# Autodesk Inventor assembly: 000 Ensamblaje hw_DAA - PCB MicroSD
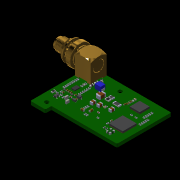
[picture p0: Inventor's stored thumbnail of the model, 180x180]
Saved by Autodesk Inventor 2018 (Build 220112000, 112)
## iProperties
Created: 2024-03-13
Part Number: 000 Ensamblaje hw_DAA - PCB MicroSD
Document SubType Name: Assembly
Designer: cda1
Author: cda1
## Documents named in this file (48)
- C:\Users\cda1\Git\DAA\items\hw_DAA\variants\BASIC\3d\000 Ensamblaje hw_DAA - PCB MicroSD.iam
- C:\Users\cda1\Git\DAA\items\hw_DAA\3d\hw_DAA - PCB MicroSD.ipt
- C:\Users\cda1\Git\DAA\items\_accessories\Componentes PCB\Tarjetero\3d_Molex\3d\47219-2001.ipt
- C:\Users\cda1\Git\DAA\items\_accessories\Cables y conectores\3d_Amphenol\3d\132203-18\132203-18.ipt
- C:\Users\cda1\Git\DAA\items\_accessories\Componentes PCB\PMIC\TPS65033000RGERQ1\TPS65033000RGERQ1.iam
- C:\Users\cda1\Git\DAA\items\_accessories\Componentes PCB\Inductor\3d_TDK\3d\NLCV32T-100K-EFRD\NLCV32T-100K-EFRD.iam
- C:\Users\cda1\Git\DAA\items\_accessories\Componentes PCB\Ferrita\3d_Murata Electronics\3d\BLM18SG121TN1D\BLM18SG121TN1D.ipt
- C:\Users\cda1\Git\DAA\items\_accessories\Componentes PCB\EMI Suppressor\3d_Murata_Electronics\BLM18AG102BH1D\BLM18AG102BH1D.ipt
- C:\Users\cda1\Git\DAA\items\_accessories\Componentes PCB\EMI Suppressor\3d_Murata_Electronics\BLM18HE152SZ1D\BLM18HE152SZ1D.ipt
- C:\Users\cda1\Git\DAA\items\_accessories\Componentes PCB\MIPI\DS90UB953TRHBTQ1\DS90UB953TRHBTQ1.iam
- C:\Users\cda1\Git\DAA\items\_accessories\Componentes PCB\FPD-Link\3d_Texas_Instruments\DS90UB954TRGZTQ1\DS90UB954TRGZTQ1.iam
- C:\Users\cda1\Git\DAA\items\_accessories\Componentes PCB\Oscilador\3d_ECS_International\ECS-2520MVQ-250-CN-TR\ECS-2520MVQ-250-CN-TR.ipt
- C:\Users\cda1\Git\DAA\items\_accessories\Componentes PCB\Capacitadores\3d_TDK\3d\CGA5L1X7R1V106K160AC.ipt
- C:\Users\cda1\Git\DAA\items\_accessories\Componentes PCB\Capacitadores\3d_TDK\3d\CGA2B3X7R1H104K050BD.ipt
- C:\Users\cda1\Git\DAA\items\_accessories\Componentes PCB\Capacitadores\3d_Taiyo Yuden\3d\EMK212BBJ106KGHT.ipt
- C:\Users\cda1\Git\DAA\items\_accessories\Componentes PCB\Resistencias\3d_Panasonic\3d\ERJ-2RKF1002X.ipt
- C:\Users\cda1\Git\DAA\items\_accessories\Componentes PCB\Resistencias\3d_Yageo\3d\AC1206FR-074R02L\AC1206FR-074R02L.ipt
- C:\Users\cda1\Git\DAA\items\_accessories\Componentes PCB\Resistencias\3d_Yageo\3d\AC0805FR-070RL.ipt
- C:\Users\cda1\Git\DAA\items\_accessories\Componentes PCB\Capacitadores\3d_Murata Electronics\3d\GRT188C81A106ME13D\GRT188C81A106ME13D.iam
- C:\Users\cda1\Git\DAA\items\_accessories\Componentes PCB\Capacitadores\3d_TDK\3d\CGA2B3X8R1H103K050BB.ipt
- C:\Users\cda1\Git\DAA\items\_accessories\Componentes PCB\Voltage-Level\3d\3d_NXP\NVT4858HK\NVT4858HK.ipt
- C:\Users\cda1\Git\DAA\items\_accessories\Componentes PCB\ESD Supressor\3d_Littlefuse\3d\AQ4020-01FTG\AQ4020-01FTG.iam
- C:\Users\cda1\Git\DAA\items\_accessories\Componentes PCB\Active-low load\3d_Texas_Instruments\TPS22910AYZVR\TPS22910AYZVR.iam
- C:\Users\cda1\Git\DAA\items\_accessories\Componentes PCB\Capacitadores\3d_Murata Electronics\3d\GRT155R61E105KE01D.ipt
- C:\Users\cda1\Git\DAA\items\_accessories\Componentes PCB\Inverter\3d_Texas Instruments\3d\SN74LVC1G04QDCKRQ1\SN74LVC1G04QDCKRQ1.iam
- C:\Users\cda1\Git\DAA\items\_accessories\Componentes PCB\Capacitadores\3d_Murata Electronics\3d\NFM18HC106D0G3L\NFM18HC106D0G3L.ipt
- C:\Users\cda1\Git\DAA\items\_accessories\Componentes PCB\Capacitadores\3d_TDK\3d\CGA3E1X7S1C225K080AC\CGA3E1X7S1C225K080AC.iam
- C:\Users\cda1\Git\DAA\items\_accessories\Componentes PCB\Resistencias\3d_Panasonic\3d\ERJ-2GE0R00X.ipt
- C:\Users\cda1\Git\DAA\items\_accessories\Componentes PCB\Capacitadores\3d_Murata Electronics\3d\GCM155R71H153KA55D\GCM155R71H153KA55D.iam
- C:\Users\cda1\Git\DAA\items\_accessories\Componentes PCB\Resistencias\3d_Panasonic\3d\ERJ-U02F4701X\ERJ-U02F4701X.iam
- C:\Users\cda1\Git\DAA\items\_accessories\Componentes PCB\Capacitadores\3d_Kemet\3d\C0402C223K5RECAUTO.ipt
- C:\Users\cda1\Git\DAA\items\_accessories\Componentes PCB\Capacitadores\3d_TDK\3d\CGA2B3X7R1H333K050BB.ipt
- C:\Users\cda1\Git\DAA\items\_accessories\Componentes PCB\Resistencias\3d_Vishay\3d\CRCW040249R9FKED\CRCW040249R9FKED.ipt
- C:\Users\cda1\Git\DAA\items\_accessories\Componentes PCB\Condensadores\3d-Murata\3d\GRT155R61A475ME13D\GRT155R61A475ME13D.iam
- C:\Users\cda1\Git\DAA\items\_accessories\Componentes PCB\Condensadores\3d-Murata\3d\GRT155C81C225KE13D.ipt
- C:\Users\cda1\Git\DAA\items\_accessories\Componentes PCB\Resistencias\3d_Vishay\3d\CRCW040240K2FKED\CRCW040240K2FKED.ipt
- C:\Users\cda1\Git\DAA\items\_accessories\Componentes PCB\Capacitadores\3d_Taiyo Yuden\3d\HMJ107BB7104KAHT.ipt
- C:\Users\cda1\Git\DAA\items\_accessories\Componentes PCB\Resistencias\3d_Genérico\RESC-1206.ipt
- C:\Users\cda1\Git\DAA\items\_accessories\Componentes PCB\Diodos\3d_Diodes Incorporated\3d\DMN2710UTQ-7\DMN2710UTQ-7.ipt
- C:\Users\cda1\Git\DAA\items\_accessories\Componentes PCB\Inductor\3d_TDK\3d\TFM201610ALMA1R0MTAA\TFM201610ALMA1R0MTAA.iam
- C:\Users\cda1\Git\DAA\items\_accessories\Componentes PCB\Inductor\3d_TDK\3d\TFM201610ALMA1R5MTAA\TFM201610ALMA1R5MTAA.iam
- C:\Users\cda1\Git\DAA\items\_accessories\Componentes PCB\Resistencias\3d_Genérico\RESC-0402.ipt
- C:\Users\cda1\Git\DAA\items\_accessories\Componentes PCB\Diodos\3d_TE_Connectivity\3d\PESD0402-140\PESD0402-140.iam
- C:\Users\cda1\Git\DAA\items\_accessories\Componentes PCB\Resistencias\3d_Genérico\RESC-0603.ipt
- C:\Users\cda1\Git\DAA\items\_accessories\Componentes PCB\Capacitadores\3d_Genérico\3d\CAPC-0402-T0.55-BN.ipt
- C:\Users\cda1\Git\DAA\items\_accessories\Componentes PCB\Transistores\3d_Diodes\3d\DMP2006UFGQ-13\DMP2006UFGQ-13.iam
- C:\Users\cda1\Git\DAA\items\_accessories\Componentes PCB\Resistencias\3d_Panasonic\3d\ERJ-2RKF33R0X.ipt
- C:\Users\cda1\Git\DAA\items\_accessories\Componentes PCB\Resistencias\3d_Genérico\RESC-0805.ipt
## Components (182 placed, 47 different names)
1. hw_DAA - PCB MicroSD:1 — Coincidencia:3, Coincidencia:4, Coincidencia:9, Coincidencia:14, Coincidencia:17, Coincidencia:18, Coincidencia:20, Coincidencia:24, Coincidencia:25, Coincidencia:34, Coincidencia:35, Coincidencia:36, Coincidencia:38, Coincidencia:39, Coincidencia:40, Coincidencia:42, Coincidencia:43, Coincidencia:50, Coincidencia:51, Coincidencia:52, Coincidencia:53, Coincidencia:54, Coincidencia:55, Coincidencia:56, Coincidencia:57, Coincidencia:59, Coincidencia:60, Coincidencia:62, Coincidencia:63, Coincidencia:64, Coincidencia:65, Coincidencia:67, Coincidencia:69, Coincidencia:70, Coincidencia:71, Coincidencia:72, Coincidencia:73, Coincidencia:74, Coincidencia:75, Coincidencia:76, Coincidencia:79, Coincidencia:95, Coincidencia:96, Coincidencia:97, Coincidencia:99, Coincidencia:101, Coincidencia:102, Coincidencia:117, Coincidencia:130, Coincidencia:131, Coincidencia:132, Coincidencia:133, Coincidencia:134, Coincidencia:135, Coincidencia:137, Coincidencia:138, Coincidencia:140, Coincidencia:141, Coincidencia:155, Coincidencia:156, Coincidencia:157, Coincidencia:158, Coincidencia:159, Coincidencia:165, Coincidencia:166, Coincidencia:167, Coincidencia:182, Coincidencia:183, Coincidencia:186, Coincidencia:187, Coincidencia:189, Coincidencia:190, Coincidencia:191, Coincidencia:192, Coincidencia:193, Coincidencia:194, Coincidencia:197, Coincidencia:198, Coincidencia:199, Coincidencia:204, Coincidencia:205, Coincidencia:206, Coincidencia:207, Coincidencia:208, Coincidencia:209, Coincidencia:210, Coincidencia:211, Ángulo:3, Ángulo:4, Coincidencia:212, Coincidencia:213, Coincidencia:214, Coincidencia:215, Coincidencia:216, Coincidencia:217, Coincidencia:218, Coincidencia:219, Coincidencia:220, Ángulo:6, Coincidencia:221, Ángulo:7, Coincidencia:222, Coincidencia:223, Ángulo:8, Ángulo:9, Coincidencia:224, Coincidencia:225, Coincidencia:226, Coincidencia:227, Coincidencia:228, Coincidencia:229, Coincidencia:230, Coincidencia:231, Coincidencia:232, Coincidencia:233, Coincidencia:234, Coincidencia:235, Coincidencia:236, Coincidencia:237, Coincidencia:238, Coincidencia:240, Coincidencia:241, Coincidencia:244, Coincidencia:245, Coincidencia:246, Coincidencia:249, Coincidencia:250, Coincidencia:251, Coincidencia:252, Coincidencia:253, Coincidencia:254, Coincidencia:255, Coincidencia:256, Coincidencia:257, Coincidencia:258, Coincidencia:259, Coincidencia:260, Coincidencia:261, Coincidencia:262, Coincidencia:263, Coincidencia:264, Coincidencia:265, Ángulo:11, Coincidencia:266, Coincidencia:267, Coincidencia:268, Coincidencia:269, Ángulo:12, Ángulo:13, Coincidencia:270, Coincidencia:271, Ángulo:16, Coincidencia:272, Coincidencia:273, Coincidencia:274, Coincidencia:275, Coincidencia:276, Coincidencia:277, Coincidencia:278, Coincidencia:279, Coincidencia:280, Coincidencia:281, Coincidencia:282, Coincidencia:283, Coincidencia:284, Coincidencia:285, Ángulo:17, Coincidencia:286, Coincidencia:287, Ángulo:18, Ángulo:19, Coincidencia:288, Coincidencia:289, Coincidencia:290, Coincidencia:291, Coincidencia:292, Coincidencia:293, Coincidencia:294, Coincidencia:295, Coincidencia:296, Coincidencia:297, Coincidencia:298, Coincidencia:299, Coincidencia:300, Coincidencia:301, Coincidencia:302, Coincidencia:303, Coincidencia:304, Coincidencia:305, Coincidencia:306, Coincidencia:307, Coincidencia:308, Coincidencia:309, Coincidencia:310, Coincidencia:311
2. 47219-2001:1 — Coincidencia:182
3. 132203-18:1 — Coincidencia:3, Coincidencia:271, Ángulo:16
4. TPS65033000RGERQ1:1 [sub-assembly] — Coincidencia:4
5. NLCV32T-100K-EFRD:1 [sub-assembly] — Coincidencia:263
6. BLM18SG121TN1D:1 — Coincidencia:9
7. BLM18AG102BH1D:2 — Coincidencia:14
8. BLM18AG102BH1D:4 — Coincidencia:17
9. BLM18AG102BH1D:5 — Coincidencia:18
10. BLM18AG102BH1D:7 — Coincidencia:20
11. BLM18HE152SZ1D:1
12. BLM18HE152SZ1D:2 — Coincidencia:268
13. BLM18HE152SZ1D:3 — Coincidencia:267
14. DS90UB953TRHBTQ1:1 [sub-assembly] — Coincidencia:24
15. DS90UB954TRGZTQ1:1 [sub-assembly] — Coincidencia:25
16. CGA5L1X7R1V106K160AC:1 — Coincidencia:264, Ángulo:17
17. CGA5L1X7R1V106K160AC:2 — Coincidencia:34
18. CGA5L1X7R1V106K160AC:3 — Coincidencia:35
19. CGA2B3X7R1H104K050BD:1 — Coincidencia:36
20. CGA2B3X7R1H104K050BD:4 — Coincidencia:39
21. CGA2B3X7R1H104K050BD:5 — Coincidencia:40
22. CGA2B3X7R1H104K050BD:6 — Coincidencia:38
23. CGA2B3X7R1H104K050BD:7 — Coincidencia:42
24. CGA2B3X7R1H104K050BD:8 — Coincidencia:43
25. CGA2B3X7R1H104K050BD:15 — Coincidencia:50
26. CGA2B3X7R1H104K050BD:16 — Coincidencia:51
27. CGA2B3X7R1H104K050BD:17 — Coincidencia:53
28. CGA2B3X7R1H104K050BD:18 — Coincidencia:52
29. CGA2B3X7R1H104K050BD:19 — Coincidencia:54
30. CGA2B3X7R1H104K050BD:20 — Coincidencia:55
31. CGA2B3X7R1H104K050BD:21 — Coincidencia:56
32. CGA2B3X7R1H104K050BD:22 — Coincidencia:57
33. CGA2B3X7R1H104K050BD:24 — Coincidencia:60
34. CGA2B3X7R1H104K050BD:25 — Coincidencia:59
35. CGA2B3X7R1H104K050BD:28 — Coincidencia:65
36. CGA2B3X7R1H104K050BD:29 — Coincidencia:64
37. CGA2B3X7R1H104K050BD:30 — Coincidencia:63
38. CGA2B3X7R1H104K050BD:31 — Coincidencia:62
39. CGA2B3X7R1H104K050BD:32 — Coincidencia:72
40. CGA2B3X7R1H104K050BD:33 — Coincidencia:71
41. CGA2B3X7R1H104K050BD:34 — Coincidencia:70
42. CGA2B3X7R1H104K050BD:35 — Coincidencia:69
43. CGA2B3X7R1H104K050BD:37 — Coincidencia:67
44. CGA2B3X7R1H104K050BD:38 — Coincidencia:76
45. CGA2B3X7R1H104K050BD:39 — Coincidencia:75
46. CGA2B3X7R1H104K050BD:40 — Coincidencia:74
47. CGA2B3X7R1H104K050BD:41 — Coincidencia:73
48. CGA2B3X7R1H104K050BD:44 — Coincidencia:79
49. CGA2B3X7R1H104K050BD:55 — Coincidencia:95
50. CGA2B3X7R1H104K050BD:56 — Coincidencia:96
51. CGA2B3X7R1H104K050BD:57 — Coincidencia:97
52. CGA2B3X7R1H104K050BD:59 — Coincidencia:99
53. CGA2B3X7R1H104K050BD:61 — Coincidencia:101
54. CGA2B3X7R1H104K050BD:62 — Coincidencia:102
55. EMK212BBJ106KGHT:1 — Coincidencia:186
56. EMK212BBJ106KGHT:2 — Coincidencia:187
57. EMK212BBJ106KGHT:3 — Coincidencia:286
58. ERJ-2RKF1002X:1 — Coincidencia:117
59. ERJ-2RKF1002X:14 — Coincidencia:130
60. ERJ-2RKF1002X:15 — Coincidencia:131
61. ERJ-2RKF1002X:16 — Coincidencia:132
62. ERJ-2RKF1002X:17 — Coincidencia:133
63. ERJ-2RKF1002X:18 — Coincidencia:134
64. ERJ-2RKF1002X:19 — Coincidencia:135
65. ERJ-2RKF1002X:21 — Coincidencia:137
66. ERJ-2RKF1002X:22 — Coincidencia:138
67. ERJ-2RKF1002X:24 — Coincidencia:140
68. ERJ-2RKF1002X:25 — Coincidencia:141
69. ERJ-2RKF1002X:38
70. ERJ-2RKF1002X:39 — Coincidencia:155
71. ERJ-2RKF1002X:40 — Coincidencia:158
72. ERJ-2RKF1002X:41 — Coincidencia:159
73. ERJ-2RKF1002X:42 — Coincidencia:156
74. ERJ-2RKF1002X:43 — Coincidencia:157
75. ERJ-2RKF1002X:49 — Coincidencia:165
76. ERJ-2RKF1002X:50 — Coincidencia:166
77. ERJ-2RKF1002X:51 — Coincidencia:167
78. CGA5L1X7R1V106K160AC:4 — Coincidencia:183, Ángulo:13
79. AC1206FR-074R02L:1 — Coincidencia:262
80. AC0805FR-070RL:1 — Coincidencia:266
81. EMK212BBJ106KGHT:4 — Coincidencia:189
82. GRT188C81A106ME13D:1 [sub-assembly] — Coincidencia:190
83. GRT188C81A106ME13D:2 [sub-assembly] — Coincidencia:191
84. GRT188C81A106ME13D:3 [sub-assembly] — Coincidencia:192
85. GRT188C81A106ME13D:4 [sub-assembly] — Coincidencia:193
86. GRT188C81A106ME13D:5 [sub-assembly] — Coincidencia:194
87. CGA2B3X8R1H103K050BB:1 — Coincidencia:197
88. CGA2B3X8R1H103K050BB:2 — Coincidencia:198
89. GRT188C81A106ME13D:6 [sub-assembly] — Coincidencia:199
90. NVT4858HK:1 — Coincidencia:204
91. AQ4020-01FTG:1 [sub-assembly] — Coincidencia:205
92. TPS22910AYZVR:1 [sub-assembly] — Coincidencia:206
93. TPS22910AYZVR:2 [sub-assembly] — Coincidencia:207
94. GRT155R61E105KE01D:1 — Coincidencia:208
95. GRT188C81A106ME13D:7 [sub-assembly] — Coincidencia:209
96. SN74LVC1G04QDCKRQ1:1 [sub-assembly] — Coincidencia:210, Coincidencia:211
97. NFM18HC106D0G3L:1 — Ángulo:3, Coincidencia:212
98. NFM18HC106D0G3L:2 — Ángulo:4, Coincidencia:213
99. EMK212BBJ106KGHT:5 — Coincidencia:215
100. EMK212BBJ106KGHT:6 — Coincidencia:214
101. CGA3E1X7S1C225K080AC:1 [sub-assembly] — Coincidencia:216, Ángulo:5
102. GRT155R61E105KE01D:2 — Coincidencia:217
103. CGA3E1X7S1C225K080AC:2 [sub-assembly] — Coincidencia:218, Ángulo:5
104. ERJ-2GE0R00X:1 — Coincidencia:219
105. ERJ-2GE0R00X:2 — Coincidencia:220, Ángulo:6
106. GCM155R71H153KA55D:1 [sub-assembly] — Coincidencia:221, Ángulo:7
107. ERJ-U02F4701X:1 [sub-assembly] — Coincidencia:222, Ángulo:9
108. ERJ-U02F4701X:2 [sub-assembly] — Coincidencia:223, Ángulo:8
109. ECS-2520MVQ-250-CN-TR:2 — Coincidencia:224
110. GCM155R71H153KA55D:2 [sub-assembly] — Coincidencia:225
111. CGA2B3X7R1H104K050BD:68 — Coincidencia:226
112. C0402C223K5RECAUTO:1 — Coincidencia:227
113. C0402C223K5RECAUTO:2 — Coincidencia:228
114. CGA2B3X7R1H333K050BB:1 — Coincidencia:229
115. CGA2B3X7R1H333K050BB:2 — Coincidencia:230
116. CRCW040249R9FKED:1 — Coincidencia:231
117. GRT155R61E105KE01D:3 — Coincidencia:232
118. GRT155R61E105KE01D:4 — Coincidencia:233
119. GRT155R61A475ME13D:1 [sub-assembly] — Coincidencia:234
120. CGA2B3X7R1H104K050BD:69 — Coincidencia:235
121. ERJ-2RKF1002X:65 — Coincidencia:236, Ángulo:18
122. GRT155C81C225KE13D:1 — Coincidencia:237, Ángulo:19
123. ERJ-2RKF1002X:66 — Coincidencia:238
124. BLM18AG102BH1D:8 — Coincidencia:240
125. CRCW040240K2FKED:1 — Coincidencia:241
126. ERJ-2GE0R00X:3 — Coincidencia:244
127. ERJ-2GE0R00X:4 — Coincidencia:246
128. ERJ-2GE0R00X:5 — Coincidencia:245
129. HMJ107BB7104KAHT:1 — Coincidencia:265, Ángulo:11
130. DMN2710UTQ-7:1 — Coincidencia:249, Coincidencia:250
131. TFM201610ALMA1R0MTAA:1 [sub-assembly] — Coincidencia:251
132. TFM201610ALMA1R5MTAA:1 [sub-assembly] — Coincidencia:252
133. TFM201610ALMA1R0MTAA:2 [sub-assembly] — Coincidencia:253
134. CGA2B3X7R1H104K050BD:70 — Coincidencia:254
135. RESC-0402:1 — Coincidencia:255
136. RESC-0402:2 — Coincidencia:256
137. ERJ-2RKF1002X:67 — Coincidencia:257
138. PESD0402-140:1 [sub-assembly] — Coincidencia:258
139. RESC-0603:1 — Coincidencia:259
140. CAPC-0402-T0.55-BN:1 — Coincidencia:260
141. RESC-0402:3 — Coincidencia:261
142. RESC-1206:2 — Coincidencia:269, Ángulo:12
143. DMP2006UFGQ-13:1 [sub-assembly] — Coincidencia:270
144. ERJ-2RKF33R0X:1 — Coincidencia:272
145. ERJ-2RKF33R0X:2 — Coincidencia:273
146. ERJ-2RKF33R0X:3 — Coincidencia:274
147. ERJ-2RKF33R0X:4 — Coincidencia:275
148. ERJ-2RKF33R0X:5 — Coincidencia:277
149. ERJ-2RKF33R0X:6 — Coincidencia:278
150. ERJ-2RKF33R0X:7 — Coincidencia:279
151. ERJ-2RKF33R0X:8 — Coincidencia:281
152. ERJ-2RKF33R0X:9 — Coincidencia:282
153. ERJ-2RKF33R0X:10 — Coincidencia:283
154. ERJ-2RKF33R0X:11 — Coincidencia:284
155. ERJ-2RKF33R0X:12 — Coincidencia:285
156. ERJ-2RKF33R0X:13 — Coincidencia:280
157. ERJ-2RKF33R0X:14 — Coincidencia:276
158. RESC-0805:1 — Coincidencia:287
159. ERJ-2RKF1002X:68 — Coincidencia:288
160. ERJ-2RKF1002X:69 — Coincidencia:289
161. ERJ-2RKF1002X:70 — Coincidencia:290
162. ERJ-2RKF1002X:71 — Coincidencia:291
163. ERJ-2RKF1002X:72 — Coincidencia:292
164. ERJ-2RKF1002X:73 — Coincidencia:293
165. ERJ-2RKF1002X:74 — Coincidencia:294
166. ERJ-2RKF1002X:75 — Coincidencia:295
167. ERJ-2RKF1002X:76 — Coincidencia:296
168. ERJ-2RKF1002X:77 — Coincidencia:297
169. ERJ-2RKF1002X:78 — Coincidencia:298
170. ERJ-2RKF1002X:79 — Coincidencia:299
171. ERJ-2GE0R00X:6 — Coincidencia:300
172. ERJ-2GE0R00X:7 — Coincidencia:301
173. ERJ-2GE0R00X:8 — Coincidencia:302
174. ERJ-2GE0R00X:9 — Coincidencia:303
175. ERJ-2GE0R00X:10 — Coincidencia:304
176. ERJ-2GE0R00X:11 — Coincidencia:305
177. ERJ-2GE0R00X:12 — Coincidencia:306
178. ERJ-2GE0R00X:13 — Coincidencia:307
179. ERJ-2GE0R00X:14 — Coincidencia:308
180. ERJ-2GE0R00X:15 — Coincidencia:309
181. ERJ-2GE0R00X:16 — Coincidencia:310
182. ERJ-2GE0R00X:17 — Coincidencia:311
## Relationships (196: Mate 182, Angle 14)
- Coincidencia:3 [Mate]: hw_DAA - PCB MicroSD:1 ↔ 132203-18:1
- Coincidencia:4 [Mate]: hw_DAA - PCB MicroSD:1 ↔ TPS65033000RGERQ1:1
- Coincidencia:9 [Mate]: hw_DAA - PCB MicroSD:1 ↔ BLM18SG121TN1D:1
- Coincidencia:14 [Mate]: hw_DAA - PCB MicroSD:1 ↔ BLM18AG102BH1D:2
- Coincidencia:17 [Mate]: hw_DAA - PCB MicroSD:1 ↔ BLM18AG102BH1D:4
- Coincidencia:18 [Mate]: hw_DAA - PCB MicroSD:1 ↔ BLM18AG102BH1D:5
- Coincidencia:20 [Mate]: hw_DAA - PCB MicroSD:1 ↔ BLM18AG102BH1D:7
- Coincidencia:24 [Mate]: hw_DAA - PCB MicroSD:1 ↔ DS90UB953TRHBTQ1:1
- Coincidencia:25 [Mate]: hw_DAA - PCB MicroSD:1 ↔ DS90UB954TRGZTQ1:1
- Coincidencia:34 [Mate]: hw_DAA - PCB MicroSD:1 ↔ CGA5L1X7R1V106K160AC:2
- Coincidencia:35 [Mate]: hw_DAA - PCB MicroSD:1 ↔ CGA5L1X7R1V106K160AC:3
- Coincidencia:36 [Mate]: hw_DAA - PCB MicroSD:1 ↔ CGA2B3X7R1H104K050BD:1
- Coincidencia:38 [Mate]: hw_DAA - PCB MicroSD:1 ↔ CGA2B3X7R1H104K050BD:6
- Coincidencia:39 [Mate]: hw_DAA - PCB MicroSD:1 ↔ CGA2B3X7R1H104K050BD:4
- Coincidencia:40 [Mate]: hw_DAA - PCB MicroSD:1 ↔ CGA2B3X7R1H104K050BD:5
- Coincidencia:42 [Mate]: hw_DAA - PCB MicroSD:1 ↔ CGA2B3X7R1H104K050BD:7
- Coincidencia:43 [Mate]: hw_DAA - PCB MicroSD:1 ↔ CGA2B3X7R1H104K050BD:8
- Coincidencia:50 [Mate]: hw_DAA - PCB MicroSD:1 ↔ CGA2B3X7R1H104K050BD:15
- Coincidencia:51 [Mate]: hw_DAA - PCB MicroSD:1 ↔ CGA2B3X7R1H104K050BD:16
- Coincidencia:52 [Mate]: hw_DAA - PCB MicroSD:1 ↔ CGA2B3X7R1H104K050BD:18
- Coincidencia:53 [Mate]: hw_DAA - PCB MicroSD:1 ↔ CGA2B3X7R1H104K050BD:17
- Coincidencia:54 [Mate]: hw_DAA - PCB MicroSD:1 ↔ CGA2B3X7R1H104K050BD:19
- Coincidencia:55 [Mate]: hw_DAA - PCB MicroSD:1 ↔ CGA2B3X7R1H104K050BD:20
- Coincidencia:56 [Mate]: hw_DAA - PCB MicroSD:1 ↔ CGA2B3X7R1H104K050BD:21
- Coincidencia:57 [Mate]: hw_DAA - PCB MicroSD:1 ↔ CGA2B3X7R1H104K050BD:22
- Coincidencia:59 [Mate]: hw_DAA - PCB MicroSD:1 ↔ CGA2B3X7R1H104K050BD:25
- Coincidencia:60 [Mate]: hw_DAA - PCB MicroSD:1 ↔ CGA2B3X7R1H104K050BD:24
- Coincidencia:62 [Mate]: hw_DAA - PCB MicroSD:1 ↔ CGA2B3X7R1H104K050BD:31
- Coincidencia:63 [Mate]: hw_DAA - PCB MicroSD:1 ↔ CGA2B3X7R1H104K050BD:30
- Coincidencia:64 [Mate]: hw_DAA - PCB MicroSD:1 ↔ CGA2B3X7R1H104K050BD:29
- Coincidencia:65 [Mate]: hw_DAA - PCB MicroSD:1 ↔ CGA2B3X7R1H104K050BD:28
- Coincidencia:67 [Mate]: hw_DAA - PCB MicroSD:1 ↔ CGA2B3X7R1H104K050BD:37
- Coincidencia:69 [Mate]: hw_DAA - PCB MicroSD:1 ↔ CGA2B3X7R1H104K050BD:35
- Coincidencia:70 [Mate]: hw_DAA - PCB MicroSD:1 ↔ CGA2B3X7R1H104K050BD:34
- Coincidencia:71 [Mate]: hw_DAA - PCB MicroSD:1 ↔ CGA2B3X7R1H104K050BD:33
- Coincidencia:72 [Mate]: hw_DAA - PCB MicroSD:1 ↔ CGA2B3X7R1H104K050BD:32
- Coincidencia:73 [Mate]: hw_DAA - PCB MicroSD:1 ↔ CGA2B3X7R1H104K050BD:41
- Coincidencia:74 [Mate]: hw_DAA - PCB MicroSD:1 ↔ CGA2B3X7R1H104K050BD:40
- Coincidencia:75 [Mate]: hw_DAA - PCB MicroSD:1 ↔ CGA2B3X7R1H104K050BD:39
- Coincidencia:76 [Mate]: hw_DAA - PCB MicroSD:1 ↔ CGA2B3X7R1H104K050BD:38
- Coincidencia:79 [Mate]: hw_DAA - PCB MicroSD:1 ↔ CGA2B3X7R1H104K050BD:44
- Coincidencia:95 [Mate]: hw_DAA - PCB MicroSD:1 ↔ CGA2B3X7R1H104K050BD:55
- Coincidencia:96 [Mate]: hw_DAA - PCB MicroSD:1 ↔ CGA2B3X7R1H104K050BD:56
- Coincidencia:97 [Mate]: hw_DAA - PCB MicroSD:1 ↔ CGA2B3X7R1H104K050BD:57
- Coincidencia:99 [Mate]: hw_DAA - PCB MicroSD:1 ↔ CGA2B3X7R1H104K050BD:59
- Coincidencia:101 [Mate]: hw_DAA - PCB MicroSD:1 ↔ CGA2B3X7R1H104K050BD:61
- Coincidencia:102 [Mate]: hw_DAA - PCB MicroSD:1 ↔ CGA2B3X7R1H104K050BD:62
- Coincidencia:117 [Mate]: hw_DAA - PCB MicroSD:1 ↔ ERJ-2RKF1002X:1
- Coincidencia:130 [Mate]: hw_DAA - PCB MicroSD:1 ↔ ERJ-2RKF1002X:14
- Coincidencia:131 [Mate]: hw_DAA - PCB MicroSD:1 ↔ ERJ-2RKF1002X:15
- Coincidencia:132 [Mate]: hw_DAA - PCB MicroSD:1 ↔ ERJ-2RKF1002X:16
- Coincidencia:133 [Mate]: hw_DAA - PCB MicroSD:1 ↔ ERJ-2RKF1002X:17
- Coincidencia:134 [Mate]: hw_DAA - PCB MicroSD:1 ↔ ERJ-2RKF1002X:18
- Coincidencia:135 [Mate]: hw_DAA - PCB MicroSD:1 ↔ ERJ-2RKF1002X:19
- Coincidencia:137 [Mate]: hw_DAA - PCB MicroSD:1 ↔ ERJ-2RKF1002X:21
- Coincidencia:138 [Mate]: hw_DAA - PCB MicroSD:1 ↔ ERJ-2RKF1002X:22
- Coincidencia:140 [Mate]: hw_DAA - PCB MicroSD:1 ↔ ERJ-2RKF1002X:24
- Coincidencia:141 [Mate]: hw_DAA - PCB MicroSD:1 ↔ ERJ-2RKF1002X:25
- Coincidencia:155 [Mate]: hw_DAA - PCB MicroSD:1 ↔ ERJ-2RKF1002X:39
- Coincidencia:156 [Mate]: hw_DAA - PCB MicroSD:1 ↔ ERJ-2RKF1002X:42
- Coincidencia:157 [Mate]: hw_DAA - PCB MicroSD:1 ↔ ERJ-2RKF1002X:43
- Coincidencia:158 [Mate]: hw_DAA - PCB MicroSD:1 ↔ ERJ-2RKF1002X:40
- Coincidencia:159 [Mate]: hw_DAA - PCB MicroSD:1 ↔ ERJ-2RKF1002X:41
- Coincidencia:165 [Mate]: hw_DAA - PCB MicroSD:1 ↔ ERJ-2RKF1002X:49
- Coincidencia:166 [Mate]: hw_DAA - PCB MicroSD:1 ↔ ERJ-2RKF1002X:50
- Coincidencia:167 [Mate]: hw_DAA - PCB MicroSD:1 ↔ ERJ-2RKF1002X:51
- Coincidencia:182 [Mate]: hw_DAA - PCB MicroSD:1 ↔ 47219-2001:1
- Coincidencia:183 [Mate]: hw_DAA - PCB MicroSD:1 ↔ CGA5L1X7R1V106K160AC:4
- Coincidencia:186 [Mate]: hw_DAA - PCB MicroSD:1 ↔ EMK212BBJ106KGHT:1
- Coincidencia:187 [Mate]: hw_DAA - PCB MicroSD:1 ↔ EMK212BBJ106KGHT:2
- Coincidencia:189 [Mate]: hw_DAA - PCB MicroSD:1 ↔ EMK212BBJ106KGHT:4
- Coincidencia:190 [Mate]: hw_DAA - PCB MicroSD:1 ↔ GRT188C81A106ME13D:1
- Coincidencia:191 [Mate]: hw_DAA - PCB MicroSD:1 ↔ GRT188C81A106ME13D:2
- Coincidencia:192 [Mate]: hw_DAA - PCB MicroSD:1 ↔ GRT188C81A106ME13D:3
- Coincidencia:193 [Mate]: hw_DAA - PCB MicroSD:1 ↔ GRT188C81A106ME13D:4
- Coincidencia:194 [Mate]: hw_DAA - PCB MicroSD:1 ↔ GRT188C81A106ME13D:5
- Coincidencia:197 [Mate]: hw_DAA - PCB MicroSD:1 ↔ CGA2B3X8R1H103K050BB:1
- Coincidencia:198 [Mate]: hw_DAA - PCB MicroSD:1 ↔ CGA2B3X8R1H103K050BB:2
- Coincidencia:199 [Mate]: hw_DAA - PCB MicroSD:1 ↔ GRT188C81A106ME13D:6
- Coincidencia:204 [Mate]: hw_DAA - PCB MicroSD:1 ↔ NVT4858HK:1
- Coincidencia:205 [Mate]: hw_DAA - PCB MicroSD:1 ↔ AQ4020-01FTG:1
- Coincidencia:206 [Mate] (0.2 mm): hw_DAA - PCB MicroSD:1 ↔ TPS22910AYZVR:1
- Coincidencia:207 [Mate] (0.2 mm): hw_DAA - PCB MicroSD:1 ↔ TPS22910AYZVR:2
- Coincidencia:208 [Mate]: hw_DAA - PCB MicroSD:1 ↔ GRT155R61E105KE01D:1
- Coincidencia:209 [Mate]: hw_DAA - PCB MicroSD:1 ↔ GRT188C81A106ME13D:7
- Coincidencia:210 [Mate]: hw_DAA - PCB MicroSD:1 ↔ SN74LVC1G04QDCKRQ1:1
- Coincidencia:211 [Mate]: hw_DAA - PCB MicroSD:1 ↔ SN74LVC1G04QDCKRQ1:1
- Ángulo:3 [Angle] (0 deg): hw_DAA - PCB MicroSD:1 ↔ NFM18HC106D0G3L:1
- Ángulo:4 [Angle] (0 deg): hw_DAA - PCB MicroSD:1 ↔ NFM18HC106D0G3L:2
- Coincidencia:212 [Mate]: hw_DAA - PCB MicroSD:1 ↔ NFM18HC106D0G3L:1
- Coincidencia:213 [Mate]: hw_DAA - PCB MicroSD:1 ↔ NFM18HC106D0G3L:2
- Coincidencia:214 [Mate]: hw_DAA - PCB MicroSD:1 ↔ EMK212BBJ106KGHT:6
- Coincidencia:215 [Mate]: hw_DAA - PCB MicroSD:1 ↔ EMK212BBJ106KGHT:5
- Coincidencia:216 [Mate]: hw_DAA - PCB MicroSD:1 ↔ CGA3E1X7S1C225K080AC:1
- Coincidencia:217 [Mate]: hw_DAA - PCB MicroSD:1 ↔ GRT155R61E105KE01D:2
- Coincidencia:218 [Mate]: hw_DAA - PCB MicroSD:1 ↔ CGA3E1X7S1C225K080AC:2
- Ángulo:5 [Angle] (0 deg): CGA3E1X7S1C225K080AC:1 ↔ CGA3E1X7S1C225K080AC:2
- Coincidencia:219 [Mate]: hw_DAA - PCB MicroSD:1 ↔ ERJ-2GE0R00X:1
- Coincidencia:220 [Mate]: hw_DAA - PCB MicroSD:1 ↔ ERJ-2GE0R00X:2
- Ángulo:6 [Angle] (0 deg): hw_DAA - PCB MicroSD:1 ↔ ERJ-2GE0R00X:2
- Coincidencia:221 [Mate]: hw_DAA - PCB MicroSD:1 ↔ GCM155R71H153KA55D:1
- Ángulo:7 [Angle] (0 deg): hw_DAA - PCB MicroSD:1 ↔ GCM155R71H153KA55D:1
- Coincidencia:222 [Mate]: hw_DAA - PCB MicroSD:1 ↔ ERJ-U02F4701X:1
- Coincidencia:223 [Mate]: hw_DAA - PCB MicroSD:1 ↔ ERJ-U02F4701X:2
- Ángulo:8 [Angle] (0 deg): hw_DAA - PCB MicroSD:1 ↔ ERJ-U02F4701X:2
- Ángulo:9 [Angle] (0 deg): hw_DAA - PCB MicroSD:1 ↔ ERJ-U02F4701X:1
- Coincidencia:224 [Mate]: hw_DAA - PCB MicroSD:1 ↔ ECS-2520MVQ-250-CN-TR:2
- Coincidencia:225 [Mate]: hw_DAA - PCB MicroSD:1 ↔ GCM155R71H153KA55D:2
- Coincidencia:226 [Mate]: hw_DAA - PCB MicroSD:1 ↔ CGA2B3X7R1H104K050BD:68
- Coincidencia:227 [Mate]: hw_DAA - PCB MicroSD:1 ↔ C0402C223K5RECAUTO:1
- Coincidencia:228 [Mate]: hw_DAA - PCB MicroSD:1 ↔ C0402C223K5RECAUTO:2
- Coincidencia:229 [Mate]: hw_DAA - PCB MicroSD:1 ↔ CGA2B3X7R1H333K050BB:1
- Coincidencia:230 [Mate]: hw_DAA - PCB MicroSD:1 ↔ CGA2B3X7R1H333K050BB:2
- Coincidencia:231 [Mate]: hw_DAA - PCB MicroSD:1 ↔ CRCW040249R9FKED:1
- Coincidencia:232 [Mate]: hw_DAA - PCB MicroSD:1 ↔ GRT155R61E105KE01D:3
- Coincidencia:233 [Mate]: hw_DAA - PCB MicroSD:1 ↔ GRT155R61E105KE01D:4
- Coincidencia:234 [Mate]: hw_DAA - PCB MicroSD:1 ↔ GRT155R61A475ME13D:1
- Coincidencia:235 [Mate]: hw_DAA - PCB MicroSD:1 ↔ CGA2B3X7R1H104K050BD:69
- Coincidencia:236 [Mate]: hw_DAA - PCB MicroSD:1 ↔ ERJ-2RKF1002X:65
- Coincidencia:237 [Mate]: hw_DAA - PCB MicroSD:1 ↔ GRT155C81C225KE13D:1
- Coincidencia:238 [Mate]: hw_DAA - PCB MicroSD:1 ↔ ERJ-2RKF1002X:66
- Coincidencia:240 [Mate]: hw_DAA - PCB MicroSD:1 ↔ BLM18AG102BH1D:8
- Coincidencia:241 [Mate]: hw_DAA - PCB MicroSD:1 ↔ CRCW040240K2FKED:1
- Coincidencia:244 [Mate]: hw_DAA - PCB MicroSD:1 ↔ ERJ-2GE0R00X:3
- Coincidencia:245 [Mate]: hw_DAA - PCB MicroSD:1 ↔ ERJ-2GE0R00X:5
- Coincidencia:246 [Mate]: hw_DAA - PCB MicroSD:1 ↔ ERJ-2GE0R00X:4
- Coincidencia:249 [Mate]: hw_DAA - PCB MicroSD:1 ↔ DMN2710UTQ-7:1
- Coincidencia:250 [Mate]: hw_DAA - PCB MicroSD:1 ↔ DMN2710UTQ-7:1
- Coincidencia:251 [Mate]: hw_DAA - PCB MicroSD:1 ↔ TFM201610ALMA1R0MTAA:1
- Coincidencia:252 [Mate]: hw_DAA - PCB MicroSD:1 ↔ TFM201610ALMA1R5MTAA:1
- Coincidencia:253 [Mate]: hw_DAA - PCB MicroSD:1 ↔ TFM201610ALMA1R0MTAA:2
- Coincidencia:254 [Mate]: hw_DAA - PCB MicroSD:1 ↔ CGA2B3X7R1H104K050BD:70
- Coincidencia:255 [Mate]: hw_DAA - PCB MicroSD:1 ↔ RESC-0402:1
- Coincidencia:256 [Mate]: hw_DAA - PCB MicroSD:1 ↔ RESC-0402:2
- Coincidencia:257 [Mate]: hw_DAA - PCB MicroSD:1 ↔ ERJ-2RKF1002X:67
- Coincidencia:258 [Mate]: hw_DAA - PCB MicroSD:1 ↔ PESD0402-140:1
- Coincidencia:259 [Mate]: hw_DAA - PCB MicroSD:1 ↔ RESC-0603:1
- Coincidencia:260 [Mate]: hw_DAA - PCB MicroSD:1 ↔ CAPC-0402-T0.55-BN:1
- Coincidencia:261 [Mate]: hw_DAA - PCB MicroSD:1 ↔ RESC-0402:3
- Coincidencia:262 [Mate]: hw_DAA - PCB MicroSD:1 ↔ AC1206FR-074R02L:1
- Coincidencia:263 [Mate]: hw_DAA - PCB MicroSD:1 ↔ NLCV32T-100K-EFRD:1
- Coincidencia:264 [Mate]: hw_DAA - PCB MicroSD:1 ↔ CGA5L1X7R1V106K160AC:1
- Coincidencia:265 [Mate]: hw_DAA - PCB MicroSD:1 ↔ HMJ107BB7104KAHT:1
- Ángulo:11 [Angle] (90 deg): hw_DAA - PCB MicroSD:1 ↔ HMJ107BB7104KAHT:1
- Coincidencia:266 [Mate]: hw_DAA - PCB MicroSD:1 ↔ AC0805FR-070RL:1
- Coincidencia:267 [Mate]: hw_DAA - PCB MicroSD:1 ↔ BLM18HE152SZ1D:3
- Coincidencia:268 [Mate]: hw_DAA - PCB MicroSD:1 ↔ BLM18HE152SZ1D:2
- Coincidencia:269 [Mate]: hw_DAA - PCB MicroSD:1 ↔ RESC-1206:2
- Ángulo:12 [Angle] (90 deg): hw_DAA - PCB MicroSD:1 ↔ RESC-1206:2
- Ángulo:13 [Angle] (0 deg): hw_DAA - PCB MicroSD:1 ↔ CGA5L1X7R1V106K160AC:4
- Coincidencia:270 [Mate]: hw_DAA - PCB MicroSD:1 ↔ DMP2006UFGQ-13:1
- Coincidencia:271 [Mate]: hw_DAA - PCB MicroSD:1 ↔ 132203-18:1
- Ángulo:16 [Angle] (0 deg): hw_DAA - PCB MicroSD:1 ↔ 132203-18:1
- Coincidencia:272 [Mate]: hw_DAA - PCB MicroSD:1 ↔ ERJ-2RKF33R0X:1
- Coincidencia:273 [Mate]: hw_DAA - PCB MicroSD:1 ↔ ERJ-2RKF33R0X:2
- Coincidencia:274 [Mate]: hw_DAA - PCB MicroSD:1 ↔ ERJ-2RKF33R0X:3
- Coincidencia:275 [Mate]: hw_DAA - PCB MicroSD:1 ↔ ERJ-2RKF33R0X:4
- Coincidencia:276 [Mate]: hw_DAA - PCB MicroSD:1 ↔ ERJ-2RKF33R0X:14
- Coincidencia:277 [Mate]: hw_DAA - PCB MicroSD:1 ↔ ERJ-2RKF33R0X:5
- Coincidencia:278 [Mate]: hw_DAA - PCB MicroSD:1 ↔ ERJ-2RKF33R0X:6
- Coincidencia:279 [Mate]: hw_DAA - PCB MicroSD:1 ↔ ERJ-2RKF33R0X:7
- Coincidencia:280 [Mate]: hw_DAA - PCB MicroSD:1 ↔ ERJ-2RKF33R0X:13
- Coincidencia:281 [Mate]: hw_DAA - PCB MicroSD:1 ↔ ERJ-2RKF33R0X:8
- Coincidencia:282 [Mate]: hw_DAA - PCB MicroSD:1 ↔ ERJ-2RKF33R0X:9
- Coincidencia:283 [Mate]: hw_DAA - PCB MicroSD:1 ↔ ERJ-2RKF33R0X:10
- Coincidencia:284 [Mate]: hw_DAA - PCB MicroSD:1 ↔ ERJ-2RKF33R0X:11
- Coincidencia:285 [Mate]: hw_DAA - PCB MicroSD:1 ↔ ERJ-2RKF33R0X:12
- Ángulo:17 [Angle] (0 deg): hw_DAA - PCB MicroSD:1 ↔ CGA5L1X7R1V106K160AC:1
- Coincidencia:286 [Mate]: hw_DAA - PCB MicroSD:1 ↔ EMK212BBJ106KGHT:3
- Coincidencia:287 [Mate]: hw_DAA - PCB MicroSD:1 ↔ RESC-0805:1
- Ángulo:18 [Angle] (0 deg): hw_DAA - PCB MicroSD:1 ↔ ERJ-2RKF1002X:65
- Ángulo:19 [Angle] (0 deg): hw_DAA - PCB MicroSD:1 ↔ GRT155C81C225KE13D:1
- Coincidencia:288 [Mate]: hw_DAA - PCB MicroSD:1 ↔ ERJ-2RKF1002X:68
- Coincidencia:289 [Mate]: hw_DAA - PCB MicroSD:1 ↔ ERJ-2RKF1002X:69
- Coincidencia:290 [Mate]: hw_DAA - PCB MicroSD:1 ↔ ERJ-2RKF1002X:70
- Coincidencia:291 [Mate]: hw_DAA - PCB MicroSD:1 ↔ ERJ-2RKF1002X:71
- Coincidencia:292 [Mate]: hw_DAA - PCB MicroSD:1 ↔ ERJ-2RKF1002X:72
- Coincidencia:293 [Mate]: hw_DAA - PCB MicroSD:1 ↔ ERJ-2RKF1002X:73
- Coincidencia:294 [Mate]: hw_DAA - PCB MicroSD:1 ↔ ERJ-2RKF1002X:74
- Coincidencia:295 [Mate]: hw_DAA - PCB MicroSD:1 ↔ ERJ-2RKF1002X:75
- Coincidencia:296 [Mate]: hw_DAA - PCB MicroSD:1 ↔ ERJ-2RKF1002X:76
- Coincidencia:297 [Mate]: hw_DAA - PCB MicroSD:1 ↔ ERJ-2RKF1002X:77
- Coincidencia:298 [Mate]: hw_DAA - PCB MicroSD:1 ↔ ERJ-2RKF1002X:78
- Coincidencia:299 [Mate]: hw_DAA - PCB MicroSD:1 ↔ ERJ-2RKF1002X:79
- Coincidencia:300 [Mate]: hw_DAA - PCB MicroSD:1 ↔ ERJ-2GE0R00X:6
- Coincidencia:301 [Mate]: hw_DAA - PCB MicroSD:1 ↔ ERJ-2GE0R00X:7
- Coincidencia:302 [Mate]: hw_DAA - PCB MicroSD:1 ↔ ERJ-2GE0R00X:8
- Coincidencia:303 [Mate]: hw_DAA - PCB MicroSD:1 ↔ ERJ-2GE0R00X:9
- Coincidencia:304 [Mate]: hw_DAA - PCB MicroSD:1 ↔ ERJ-2GE0R00X:10
- Coincidencia:305 [Mate]: hw_DAA - PCB MicroSD:1 ↔ ERJ-2GE0R00X:11
- Coincidencia:306 [Mate]: hw_DAA - PCB MicroSD:1 ↔ ERJ-2GE0R00X:12
- Coincidencia:307 [Mate]: hw_DAA - PCB MicroSD:1 ↔ ERJ-2GE0R00X:13
- Coincidencia:308 [Mate]: hw_DAA - PCB MicroSD:1 ↔ ERJ-2GE0R00X:14
- Coincidencia:309 [Mate]: hw_DAA - PCB MicroSD:1 ↔ ERJ-2GE0R00X:15
- Coincidencia:310 [Mate]: hw_DAA - PCB MicroSD:1 ↔ ERJ-2GE0R00X:16
- Coincidencia:311 [Mate]: hw_DAA - PCB MicroSD:1 ↔ ERJ-2GE0R00X:17
